# Autodesk Inventor assembly: Ensamblaje2
(part 2 of 3)
522. Tornillo Allen cabeza botón M4x10mm:7 — Insertar:733
523. Tornillo Allen cabeza botón M4x10mm:8 — Insertar:734
524. Tornillo Allen cabeza botón M4x20mm:43 — Insertar:747
525. Tornillo Allen cabeza botón M4x20mm:44 — Insertar:748
526. Tornillo Allen cabeza botón M4x20mm:45 — Insertar:750
527. Tornillo Allen cabeza botón M4x20mm:46 — Insertar:749
528. Tornillo Allen cabeza botón M4x20mm:47 — Insertar:739
529. Tornillo Allen cabeza botón M4x20mm:48 — Insertar:740
530. Tornillo Allen cabeza botón M4x20mm:49 — Insertar:741
531. Tornillo Allen cabeza botón M4x20mm:50 — Insertar:742
532. Arandela Plana Tipo A DIN 125 - M4:42 — Insertar:739, Insertar:743
533. Arandela Plana Tipo A DIN 125 - M4:43 — Insertar:740, Insertar:744
534. Arandela Plana Tipo A DIN 125 - M4:44 — Insertar:741, Insertar:745
535. Arandela Plana Tipo A DIN 125 - M4:45 — Insertar:742, Insertar:746
536. Puerta Frontal:1 — Coincidencia:409, Coincidencia:410, Insertar:826, Insertar:827, Insertar:842, Insertar:843, Insertar:844, Insertar:845, Ángulo:7
537. Puerta Lateral Derecha:1 — Insertar:755, Insertar:756, Insertar:806, Insertar:807, Insertar:808, Insertar:809, Insertar:810, Insertar:811, Ángulo:8
538. Puerta de Inspección:1 — Insertar:757, Coincidencia:407, Coincidencia:408, Insertar:800, Insertar:801, Insertar:802, Insertar:803, Insertar:804, Insertar:805, Ángulo:4
539. Tornillo Allen cabeza botón M4x10mm:15 — Insertar:764
540. Tornillo Allen cabeza botón M4x10mm:16 — Insertar:765
541. Tornillo Allen cabeza botón M4x10mm:17 — Insertar:766
542. Tornillo Allen cabeza botón M4x10mm:18 — Insertar:769
543. Tornillo Allen cabeza botón M4x10mm:19 — Insertar:768
544. Tornillo Allen cabeza botón M4x10mm:20 — Insertar:767
545. Tornillo Allen cabeza botón M4x10mm:23 — Insertar:772
546. Tornillo Allen cabeza botón M4x10mm:24 — Insertar:773
547. Tornillo Allen cabeza botón M4x10mm:25 — Insertar:775
548. Tornillo Allen cabeza botón M4x10mm:26 — Insertar:777
549. Tornillo Allen cabeza botón M4x10mm:27 — Insertar:776
550. Tornillo Allen cabeza botón M4x10mm:28 — Insertar:774
551. ISO 4032 M4:3 — Insertar:790
552. ISO 4032 M4:4 — Insertar:791
553. ISO 4032 M4:5 — Insertar:792
554. ISO 4032 M4:6 — Insertar:793
555. ISO 4032 M4:7 — Insertar:794
556. ISO 4032 M4:8 — Insertar:795
557. ISO 4032 M4:9 — Insertar:796
558. ISO 4032 M4:10 — Insertar:797
559. ISO 4032 M4:11 — Insertar:798
560. ISO 4032 M4:12 — Insertar:799
561. ISO 4032 M4:13 — Insertar:800
562. ISO 4032 M4:14 — Insertar:801
563. ISO 4032 M4:15 — Insertar:802
564. ISO 4032 M4:16 — Insertar:803
565. ISO 4032 M4:17 — Insertar:804
566. ISO 4032 M4:18 — Insertar:805
567. ISO 4032 M4:19 — Insertar:806
568. ISO 4032 M4:20 — Insertar:807
569. ISO 4032 M4:21 — Insertar:808
570. ISO 4032 M4:22 — Insertar:809
571. ISO 4032 M4:23 — Insertar:810
572. ISO 4032 M4:24 — Insertar:811
573. Arandela Plana Tipo A DIN 125 - M4:46 — Insertar:782, Insertar:797
574. Arandela Plana Tipo A DIN 125 - M4:47 — Insertar:781, Insertar:799
575. Arandela Plana Tipo A DIN 125 - M4:48 — Insertar:789, Insertar:795
576. Arandela Plana Tipo A DIN 125 - M4:49 — Insertar:780, Insertar:798
577. Arandela Plana Tipo A DIN 125 - M4:50 — Insertar:784, Insertar:790
578. Arandela Plana Tipo A DIN 125 - M4:51 — Insertar:785, Insertar:791
579. Arandela Plana Tipo A DIN 125 - M4:52 — Insertar:783, Insertar:796
580. Arandela Plana Tipo A DIN 125 - M4:53 — Insertar:786, Insertar:792
581. Arandela Plana Tipo A DIN 125 - M4:54 — Insertar:787, Insertar:793
582. Arandela Plana Tipo A DIN 125 - M4:55 — Insertar:788, Insertar:794
583. Tornillo allen cabeza boton M5x10mm:1 — Insertar:812
584. Tornillo allen cabeza boton M5x10mm:2 — Insertar:813
585. Tornillo allen cabeza boton M5x10mm:3 — Insertar:814
586. Tornillo allen cabeza boton M5x10mm:4 — Insertar:815
587. Soporte para culata carcasa:1 — Insertar:817, Insertar:818
588. Soporte para culata carcasa:2 — Insertar:816, Insertar:819
589. Tornillo Allen cabeza botón M4x10mm:55 — Insertar:829
590. Tornillo Allen cabeza botón M4x10mm:56 — Insertar:828
591. ISO 4032 M4:25 — Insertar:830
592. ISO 4032 M4:26 — Insertar:831
593. Tornillo Allen cabeza botón M4x16mm:1 — Insertar:840
594. Tornillo Allen cabeza botón M4x16mm:2 — Insertar:839
595. Tornillo Allen cabeza botón M4x16mm:3 — Insertar:838
596. Tornillo Allen cabeza botón M4x16mm:4 — Insertar:837
597. Tornillo Allen cabeza botón M4x16mm:5 — Insertar:836
598. Tornillo Allen cabeza botón M4x16mm:6 — Insertar:841
599. Tornillo Allen cabeza botón M4x16mm:7 — Insertar:832
600. Tornillo Allen cabeza botón M4x16mm:8 — Insertar:833
601. Tornillo Allen cabeza botón M4x16mm:9 — Insertar:834
602. Tornillo Allen cabeza botón M4x16mm:10 — Insertar:835
603. ISO 4032 M4:27 — Insertar:842
604. ISO 4032 M4:28 — Insertar:843
605. ISO 4032 M4:29 — Insertar:844
606. ISO 4032 M4:30 — Insertar:845
607. Tornillo Allen cabeeza botón M3x8mm:33 — Insertar:846, Coincidencia:415
608. Tornillo Allen cabeeza botón M3x8mm:34 — Insertar:847, Coincidencia:417
609. ISO 4032 M2:1 — Coincidencia:411, Coincidencia:412
610. ISO 4032 M2:2 — Coincidencia:413, Coincidencia:414
611. ISO 4032 M3:1 — Coincidencia:415, Coincidencia:416
612. ISO 4032 M3:2 — Coincidencia:417, Coincidencia:418
613. ISO 4032 M2:3 — Coincidencia:419, Coincidencia:420
614. ISO 4032 M2:4 — Coincidencia:421, Coincidencia:422
615. Kit de sujecion 2:2 — Insertar:854, Insertar:855, Insert:858, Insert:859
616. Kit sugecion 1:1 — Insertar:852, Insertar:853, Insert:856, Insert:857
617. Eslabon cadena portacable:1 — Coincidencia:423, Nivelación:60
618. Tornillo Allen cabeeza botón M3x8mm:35 — Insert:856
619. Tornillo Allen cabeeza botón M3x8mm:36 — Insert:857
620. Tornillo Allen cabeeza botón M3x16mm:1 — Insert:858
621. Tornillo Allen cabeeza botón M3x16mm:2 — Insert:859
622. ISO 4032 M3:3 — Insert:860
623. ISO 4032 M3:4 — Insert:861
## Relationships (824: Insert 566, Mate 220, Flush 35, Angle 3)
- Coincidencia:4 [Mate]: Culata:1 ↔ Lateral:1
- Insertar:1 (-20 mm): Soporte para Patas Regulables:4 ↔ Pata regulable M6:1
- Insertar:2 (-20 mm): Soporte para Patas Regulables:1 ↔ Pata regulable M6:2
- Insertar:3 (-20 mm): Soporte para Patas Regulables:2 ↔ Pata regulable M6:3
- Insertar:4 (-20 mm): Soporte para Patas Regulables:3 ↔ Pata regulable M6:4
- Coincidencia:21 [Mate]: Frente:1 ↔ Buje para Tornillo:1
- Coincidencia:22 [Mate]: Frente:1 ↔ Buje para Tornillo:1
- Coincidencia:37 [Mate]: Columna Izquierda:1 ↔ Travesaño Estructural:1
- Coincidencia:40 [Mate]: Columna Derecha:1 ↔ Travesaño Estructural:1
- Coincidencia:41 [Mate]: Columna Derecha:1 ↔ Travesaño Estructural:1
- Coincidencia:42 [Mate]: Columna Izquierda:1 ↔ Travesaño Estructural:1
- Coincidencia:43 [Mate]: Columna Izquierda:1 ↔ Travesaño Estructural:1
- Coincidencia:44 [Mate]: Columna Derecha:1 ↔ Travesaño Estructural:1
- Coincidencia:45 [Mate]: Columna Izquierda:1 ↔ Guías de Vínculo Cabezal:2
- Nivelación:7 [Flush]: Columna Derecha:1 ↔ Guías de Vínculo Cabezal:2
- Coincidencia:46 [Mate]: Columna Derecha:1 ↔ Guías de Vínculo Cabezal:1
- Nivelación:8 [Flush]: Columna Derecha:1 ↔ Guías de Vínculo Cabezal:1
- Coincidencia:47 [Mate]: Columna Izquierda:1 ↔ Buje para Tornillo:2
- Coincidencia:48 [Mate]: Columna Izquierda:1 ↔ Buje para Tornillo:2
- Insertar:17: Tornillo de Vínculo Cabezal:1 ↔ Buje para Tornillo:2
- Coincidencia:53 [Mate]: Vertical Vìnculo Cabezal:1 ↔ Piso, Vínculo Cabezal:1
- Coincidencia:54 [Mate]: Vertical Vìnculo Cabezal:1 ↔ Piso, Vínculo Cabezal:1
- Coincidencia:55 [Mate]: Vertical Vìnculo Cabezal:1 ↔ Techo, Vínculo Cabezal:1
- Coincidencia:56 [Mate]: Vertical Vìnculo Cabezal:1 ↔ Techo, Vínculo Cabezal:1
- Coincidencia:61 [Mate]: Guías de Vínculo Cabezal:2 ↔ Buje para Guía:8
- Coincidencia:62 [Mate]: Guías de Vínculo Cabezal:2 ↔ Buje para Guía:7
- Coincidencia:63 [Mate]: Guías de Vínculo Cabezal:2 ↔ Separador de Bujes:2
- Coincidencia:64 [Mate]: Guías de Vínculo Cabezal:1 ↔ Buje para Guía:5
- Coincidencia:65 [Mate]: Guías de Vínculo Cabezal:1 ↔ Separador de Bujes:1
- Coincidencia:66 [Mate]: Guías de Vínculo Cabezal:1 ↔ Buje para Guía:6
- Coincidencia:67 [Mate]: Buje para Guía:8 ↔ Separador de Bujes:2
- Coincidencia:68 [Mate]: Buje para Guía:7 ↔ Separador de Bujes:2
- Coincidencia:69 [Mate]: Buje para Guía:6 ↔ Separador de Bujes:1
- Coincidencia:70 [Mate]: Buje para Guía:5 ↔ Separador de Bujes:1
- Coincidencia:71 [Mate]: Guías de Vínculo Cabezal:2 ↔ Tapa para Buje:4
- Coincidencia:72 [Mate]: Guías de Vínculo Cabezal:2 ↔ Tapa para Buje:1
- Coincidencia:73 [Mate]: Guías de Vínculo Cabezal:1 ↔ Tapa para Buje:3
- Coincidencia:74 [Mate]: Guías de Vínculo Cabezal:1 ↔ Tapa para Buje:2
- Coincidencia:79 [Mate]: Piso, Vínculo Cabezal:1 ↔ Buje para Tornillo:3
- Coincidencia:80 [Mate]: Piso, Vínculo Cabezal:1 ↔ Buje para Tornillo:3
- Insertar:24: Buje para Tornillo:3 ↔ Tornillo de Soporte de Motor:1
- Insertar:35: Lateral:1 ↔ Tornillo allen cabeza cilindrica M6x20mm:16
- Insertar:36: Lateral:1 ↔ Tornillo allen cabeza cilindrica M6x20mm:17
- Insertar:37: Lateral:1 ↔ Tornillo allen cabeza cilindrica M6x20mm:15
- Insertar:38: Lateral:1 ↔ Tornillo allen cabeza cilindrica M6x20mm:10
- Insertar:71: Lateral:1 ↔ Soporte para Patas Regulables:4
- Insertar:72: Lateral:1 ↔ Soporte para Patas Regulables:1
- Coincidencia:89 [Mate]: Lateral:1 ↔ Soporte para Patas Regulables:4
- Coincidencia:90 [Mate]: Lateral:1 ↔ Soporte para Patas Regulables:1
- Insertar:73: Soporte para Patas Regulables:2 ↔ Tornillo Allen cabeza fresada M4x16mm:8
- Insertar:74: Soporte para Patas Regulables:2 ↔ Tornillo Allen cabeza fresada M4x16mm:4
- Insertar:75: Soporte para Patas Regulables:3 ↔ Tornillo Allen cabeza fresada M4x16mm:7
- Insertar:76: Soporte para Patas Regulables:3 ↔ Tornillo Allen cabeza fresada M4x16mm:6
- Insertar:77: Soporte para Patas Regulables:1 ↔ Tornillo Allen cabeza fresada M4x16mm:1
- Insertar:78: Soporte para Patas Regulables:1 ↔ Tornillo Allen cabeza fresada M4x16mm:2
- Insertar:79: Soporte para Patas Regulables:4 ↔ Tornillo Allen cabeza fresada M4x16mm:3
- Insertar:80: Soporte para Patas Regulables:4 ↔ Tornillo Allen cabeza fresada M4x16mm:5
- Insertar:82: Nema 17:1 ↔ Techo Espaciador Sub. Inferior:1
- Insertar:83: Tornillo Allen cabeza cilindrica M4x16mm:1 ↔ Techo Espaciador Sub. Inferior:1
- Insertar:84: Tornillo Allen cabeza cilindrica M4x16mm:3 ↔ Techo Espaciador Sub. Inferior:1
- Insertar:85: Tornillo Allen cabeza cilindrica M4x16mm:6 ↔ Techo Espaciador Sub. Inferior:1
- Insertar:86: Tornillo Allen cabeza cilindrica M4x16mm:2 ↔ Techo Espaciador Sub. Inferior:1
- Coincidencia:91 [Mate]: Culata:1 ↔ Espaciador Sub Inferior:2
- Coincidencia:92 [Mate]: Culata:1 ↔ Espaciador Sub Inferior:1
- Coincidencia:93 [Mate]: Culata:1 ↔ Espaciador Sub Inferior:1
- Coincidencia:94 [Mate]: Culata:1 ↔ Espaciador Sub Inferior:1
- Coincidencia:95 [Mate]: Culata:1 ↔ Espaciador Sub Inferior:2
- Coincidencia:96 [Mate]: Culata:1 ↔ Espaciador Sub Inferior:2
- Coincidencia:97 [Mate]: Espaciador Sub Inferior:1 ↔ Techo Espaciador Sub. Inferior:1
- Insertar:91: Espaciador Sub Inferior:1 ↔ Techo Espaciador Sub. Inferior:1
- Coincidencia:99 [Mate]: Tornillo Allen cabeza cilindrica M4x16mm:1 ↔ Nema 17:1
- Insertar:100: Arandela Grower m6:13 ↔ Tornillo Allen cabeza botón M6x20mm:3
- Insertar:103: Arandela Grower m6:9 ↔ Tornillo Allen cabeza botón M6x20mm:8
- Insertar:107: Arandela Grower m6:10 ↔ Tornillo Allen cabeza botón M6x20mm:4
- Insertar:109: Arandela Grower m6:7 ↔ Tornillo Allen cabeza botón M6x20mm:6
- Insertar:122: Arandela Grower m6:11 ↔ Tornillo Allen cabeza botón M6x20mm:11
- Insertar:123: Arandela Grower m6:14 ↔ Tornillo Allen cabeza botón M6x20mm:21
- Insertar:124: Arandela Grower m6:8 ↔ Tornillo Allen cabeza botón M6x20mm:12
- Insertar:125: Arandela Grower m6:12 ↔ Tornillo Allen cabeza botón M6x20mm:20
- Insertar:126: Columna Izquierda:1 ↔ Arandela Grower m6:14
- Insertar:127: Columna Izquierda:1 ↔ Arandela Grower m6:11
- Insertar:128: Columna Derecha:1 ↔ Arandela Grower m6:8
- Insertar:129: Columna Derecha:1 ↔ Arandela Grower m6:12
- Insertar:138: Vertical Vìnculo Cabezal:1 ↔ Tornillo Allen cabeza botón M6x20mm:18
- Insertar:139: Vertical Vìnculo Cabezal:1 ↔ Tornillo Allen cabeza botón M6x20mm:25
- Insertar:140: Vertical Vìnculo Cabezal:1 ↔ Tornillo Allen cabeza botón M6x20mm:24
- Insertar:141: Vertical Vìnculo Cabezal:1 ↔ Tornillo Allen cabeza botón M6x20mm:28
- Insertar:142: Vertical Vìnculo Cabezal:1 ↔ Tornillo Allen cabeza botón M6x20mm:27
- Insertar:143: Vertical Vìnculo Cabezal:1 ↔ Tornillo Allen cabeza botón M6x20mm:23
- Insertar:144: Vertical Vìnculo Cabezal:1 ↔ Tornillo Allen cabeza botón M6x20mm:22
- Insertar:145: Vertical Vìnculo Cabezal:1 ↔ Tornillo Allen cabeza botón M6x20mm:26
- Insertar:148: Tapa para Buje:1 ↔ Tornillo Allen cabeeza botón M3x8mm:7
- Insertar:149: Tapa para Buje:1 ↔ Tornillo Allen cabeeza botón M3x8mm:8
- Insertar:150: Tapa para Buje:3 ↔ Tornillo Allen cabeeza botón M3x8mm:2
- Insertar:151: Tapa para Buje:3 ↔ Tornillo Allen cabeeza botón M3x8mm:6
- Insertar:152: Tapa para Buje:4 ↔ Tornillo Allen cabeeza botón M3x8mm:3
- Insertar:153: Tapa para Buje:4 ↔ Tornillo Allen cabeeza botón M3x8mm:1
- Insertar:154: Tapa para Buje:2 ↔ Tornillo Allen cabeeza botón M3x8mm:4
- Insertar:155: Tapa para Buje:2 ↔ Tornillo Allen cabeeza botón M3x8mm:5
- Coincidencia:105 [Mate]: Techo, Vínculo Cabezal:1 ↔ Espaciador Izquierdo:1
- Coincidencia:106 [Mate]: Techo, Vínculo Cabezal:1 ↔ Espaciador Izquierdo:1
- Coincidencia:107 [Mate]: Techo, Vínculo Cabezal:1 ↔ Espaciador Izquierdo:1
- Coincidencia:108 [Mate]: Techo, Vínculo Cabezal:1 ↔ Espaciador Derecho:1
- Coincidencia:109 [Mate]: Techo, Vínculo Cabezal:1 ↔ Espaciador Derecho:1
- Coincidencia:110 [Mate]: Techo, Vínculo Cabezal:1 ↔ Espaciador Derecho:1
- Coincidencia:111 [Mate]: Espaciador Izquierdo:1 ↔ Techo Espaciador:1
- Coincidencia:112 [Mate]: Espaciador Derecho:1 ↔ Techo Espaciador:1
- Coincidencia:113 [Mate]: Espaciador Derecho:1 ↔ Techo Espaciador:1
- Coincidencia:114 [Mate]: Espaciador Izquierdo:1 ↔ Techo Espaciador:1
- Coincidencia:115 [Mate]: Nema 17:3 ↔ Acople de Motor PAP:3
- Insertar:165: Techo Espaciador:1 ↔ Tornillo Allen cabeza cilindrica M4x20mm:3
- Insertar:166: Techo Espaciador:1 ↔ Tornillo Allen cabeza cilindrica M4x20mm:2
- Insertar:167: Techo Espaciador:1 ↔ Tornillo Allen cabeza cilindrica M4x20mm:1
- Insertar:168: Techo Espaciador:1 ↔ Tornillo Allen cabeza cilindrica M4x20mm:4
- Insertar:169: Nema 17:3 ↔ Techo Espaciador:1
- Insertar:170: Columna Derecha:1 ↔ Tornillo Allen cabeza botón M4x20mm:5
- Insertar:172: Columna Derecha:1 ↔ Tornillo Allen cabeza botón M4x20mm:4
- Insertar:173: Columna Derecha:1 ↔ Tornillo Allen cabeza botón M4x20mm:3
- Coincidencia:116 [Mate]: Columna Derecha:1 ↔ Nema 17:2
- Insertar:174: Columna Derecha:1 ↔ Nema 17:2
- Insertar:175: Columna Derecha:1 ↔ Nema 17:2
- Coincidencia:117 [Mate]: Tornillo de Vínculo Cabezal:1 ↔ Nema 17:2
- Insertar:176: Tornillo de Vínculo Cabezal:1 ↔ Acople de Motor PAP:2
- Coincidencia:118 [Mate]: Vertical Vìnculo Cabezal:1 ↔ Bloque - Vinculo Cabezal:1
- Coincidencia:119 [Mate]: Bloque - Vinculo Cabezal:1 ↔ Techo, Vínculo Cabezal:1
- Coincidencia:120 [Mate]: Vertical Vìnculo Cabezal:1 ↔ Bloque - Vinculo Cabezal:1
- Insertar:177: Bloque - Vinculo Cabezal:1 ↔ Buje para Guía:7
- Insertar:178: Bloque - Vinculo Cabezal:1 ↔ Buje para Guía:5
- Insertar:179: Bloque - Vinculo Cabezal:1 ↔ Tapa para Buje:4
- Insertar:180: Bloque - Vinculo Cabezal:1 ↔ Tapa para Buje:2
- Insertar:181: Bloque - Vinculo Cabezal:1 ↔ Tapa para Buje:1
- Insertar:182: Bloque - Vinculo Cabezal:1 ↔ Tapa para Buje:3
- Insertar:185: Techo Espaciador:1 ↔ Tornillo Allen cabeza cilindrica M4x45mm:3
- Insertar:186: Techo Espaciador:1 ↔ Tornillo Allen cabeza cilindrica M4x45mm:1
- Insertar:187: Techo Espaciador:1 ↔ Tornillo Allen cabeza cilindrica M4x45mm:4
- Coincidencia:125 [Mate]: Bloque - Vinculo Cabezal:1 ↔ Acople de Motor PAP:2
- Coincidencia:126 [Mate]: Columna Izquierda:1 ↔ Soporte de Final de Carrera - Eje X:1
- Coincidencia:127 [Mate]: Columna Izquierda:1 ↔ Soporte de Final de Carrera - Eje X:1
- Coincidencia:128 [Mate]: Columna Izquierda:1 ↔ Soporte de Final de Carrera - Eje X:1
- Coincidencia:129 [Mate]: Final de Carrera:2 ↔ Soporte de Final de Carrera - Eje X:1
- Coincidencia:130 [Mate]: Final de Carrera:2 ↔ Soporte de Final de Carrera - Eje X:1
- Coincidencia:131 [Mate]: Final de Carrera:2 ↔ Soporte de Final de Carrera - Eje X:1
- Coincidencia:139 [Mate]: Bloque - Vinculo Cabezal:1 ↔ Final de Carrera:2
- Insertar:201: Columna Izquierda:1 ↔ Arandela Grower m6:21
- Insertar:202: Columna Izquierda:1 ↔ Arandela Grower m6:20
- Insertar:203: Columna Izquierda:1 ↔ Arandela Grower m6:19
- Insertar:204: Columna Izquierda:1 ↔ Arandela Grower m6:24
- Insertar:205: Columna Derecha:1 ↔ Arandela Grower m6:23
- Insertar:206: Columna Derecha:1 ↔ Arandela Grower m6:17
- Insertar:207: Columna Derecha:1 ↔ Arandela Grower m6:22
- Insertar:208: Columna Derecha:1 ↔ Arandela Grower m6:18
- Insertar:213: Soporte de Final de Carrera - Eje X:1 ↔ Tornillo Allen cabeeza botón M3x8mm:10
- Insertar:214: Soporte de Final de Carrera - Eje X:1 ↔ Tornillo Allen cabeeza botón M3x8mm:9
- Insertar:217: Techo Espaciador:1 ↔ Tornillo Allen cabeza cilindrica M4x45mm:4
- Insertar:218: Techo Espaciador:1 ↔ Tornillo Allen cabeza cilindrica M4x45mm:1
- Insertar:219: Techo Espaciador:1 ↔ Tornillo Allen cabeza cilindrica M4x45mm:2
- Insertar:220: Techo Espaciador:1 ↔ Tornillo Allen cabeza cilindrica M4x45mm:3
- Coincidencia:148 [Mate]: Culata:1 ↔ Tornillo allen cabeza cilindrica M6x20mm:15
- Nivelación:12 [Flush]: Frente:1 ↔ Lateral:1
- Nivelación:16 [Flush]: Frente:1 ↔ Lateral:2
- Nivelación:17 [Flush]: Frente:1 ↔ Lateral:2
- Coincidencia:154 [Mate]: Frente:1 ↔ Lateral:2
- Insertar:234: Lateral:2 ↔ Tornillo allen cabeza cilindrica M6x20mm:20
- Insertar:235: Lateral:2 ↔ Tornillo allen cabeza cilindrica M6x20mm:5
- Insertar:236: Frente:1 ↔ Lateral:1
- Insertar:237: Lateral:2 ↔ Columna Derecha:1
- Insertar:238: Lateral:2 ↔ Columna Derecha:1
- Insertar:239: Lateral:2 ↔ Soporte para Patas Regulables:2
- Coincidencia:155 [Mate]: Lateral:2 ↔ Tornillo Allen cabeza fresada M4x16mm:4
- Insertar:254: Lateral:2 ↔ Soporte para Patas Regulables:3
- Coincidencia:170 [Mate]: Lateral:2 ↔ Soporte para Patas Regulables:3
- Coincidencia:171 [Mate]: Bloque - Vinculo Cabezal:1 ↔ Tornillo Gusano Allen M3x16mm:1
- Coincidencia:172 [Mate]: Bloque - Vinculo Cabezal:1 ↔ Tornillo Gusano Allen M3x16mm:2
- Coincidencia:173 [Mate]: Tornillo de Vínculo Cabezal:1 ↔ Tuerca de mesa:3
- Insertar:255 (10 mm): Bloque - Vinculo Cabezal:1 ↔ Tuerca de mesa:3
- Coincidencia:174 [Mate]: Bloque - Vinculo Cabezal:1 ↔ Tuerca de mesa:3
- Nivelación:18 [Flush]: Tornillo Gusano Allen M3x16mm:1 ↔ Tuerca de mesa:3
- Nivelación:19 [Flush]: Tornillo Gusano Allen M3x16mm:2 ↔ Tuerca de mesa:3
- Insertar:257: Tornillo Gusano Allen M3x16mm:4 ↔ Tuerca de mesa:2
- Coincidencia:180 [Mate]: Guías de Soporte de Motor:1 ↔ Buje de Soporte de Motor:2
- Insertar:266: Buje de Soporte de Motor:1 ↔ Tornillo Allen cabeeza botón M3x8mm:11
- Coincidencia:182 [Mate]: Guías de Soporte de Motor:2 ↔ Buje de Soporte de Motor:5
- Insertar:268: Buje de Soporte de Motor:2 ↔ Tornillo Allen cabeeza botón M3x8mm:13
- Insertar:270: Tornillo Allen cabeeza botón M3x8mm:12 ↔ Buje de Soporte de Motor:6
- Insertar:271: Buje de Soporte de Motor:5 ↔ Tornillo Allen cabeeza botón M3x8mm:16
- Nivelación:20 [Flush]: Culata:1 ↔ Acople de Motor PAP:1
- Coincidencia:186 [Mate]: Culata:1 ↔ Acople de Motor PAP:1
- Insertar:278: Tornillo de mesa:1 ↔ Buje para Tornillo:1
- Insertar:279: Techo, Vínculo Cabezal:1 ↔ Guías de Soporte de Motor:2
- Insertar:280: Techo, Vínculo Cabezal:1 ↔ Guías de Soporte de Motor:1
- Insertar:285: Frente:1 ↔ Guias de mesa:1
- Coincidencia:190 [Mate]: Guias de mesa:1 ↔ Buje para Guía:2
- Coincidencia:193 [Mate]: Frente:1 ↔ Guias de mesa:2
- Insertar:286: Frente:1 ↔ Guias de mesa:2
- Coincidencia:194 [Mate]: Guias de mesa:2 ↔ Buje para Guía:4
- Coincidencia:197 [Mate]: Mesa:1 ↔ Soporte de Buje:4
- Coincidencia:198 [Mate]: Mesa:1 ↔ Soporte de Buje:3
- Coincidencia:200 [Mate]: Mesa:1 ↔ Soporte de Buje:4
- Coincidencia:203 [Mate]: Mesa:1 ↔ Soporte de Buje:3
- Coincidencia:205 [Mate]: Mesa:1 ↔ Soporte de Buje:4
- Coincidencia:206 [Mate]: Mesa:1 ↔ Soporte de Buje:3
- Coincidencia:208 [Mate]: Mesa:1 ↔ Soporte de tuerca de mesa:1
- Coincidencia:209 [Mate]: Mesa:1 ↔ Soporte de tuerca de mesa:1
- Coincidencia:210 [Mate]: Mesa:1 ↔ Soporte de tuerca de mesa:1
- Coincidencia:211 [Mate]: Soporte de Buje:1 ↔ Buje para Guía:2
- Coincidencia:212 [Mate]: Guias de mesa:1 ↔ Buje para Guía:1
- Coincidencia:213 [Mate]: Soporte de Buje:2 ↔ Buje para Guía:1
- Nivelación:21 [Flush]: Soporte de Buje:2 ↔ Buje para Guía:1
- Nivelación:22 [Flush]: Soporte de Buje:1 ↔ Buje para Guía:2
- Coincidencia:214 [Mate]: Soporte de Buje:4 ↔ Buje para Guía:4
- Nivelación:23 [Flush]: Soporte de Buje:4 ↔ Buje para Guía:4
- Coincidencia:215 [Mate]: Soporte de Buje:3 ↔ Buje para Guía:3
- Nivelación:24 [Flush]: Soporte de Buje:3 ↔ Buje para Guía:3
- Coincidencia:216 [Mate]: Tornillo de mesa:1 ↔ Soporte de tuerca de mesa:1
- Coincidencia:217 [Mate]: Mesa:1 ↔ Soporte de Buje:2
- Coincidencia:218 [Mate]: Mesa:1 ↔ Soporte de Buje:1
- Insertar:287: Soporte de Buje:3 ↔ Tornillo Allen cabeza cilindrica M4x30mm:6
- Insertar:288: Soporte de Buje:3 ↔ Tornillo Allen cabeza cilindrica M4x30mm:9
- Insertar:289: Soporte de Buje:3 ↔ Tornillo Allen cabeza cilindrica M4x30mm:18
- Insertar:290: Soporte de Buje:3 ↔ Tornillo Allen cabeza cilindrica M4x30mm:1
- Insertar:291: Soporte de Buje:2 ↔ Tornillo Allen cabeza cilindrica M4x30mm:2
- Insertar:292: Soporte de Buje:2 ↔ Tornillo Allen cabeza cilindrica M4x30mm:16
- Insertar:293: Soporte de Buje:2 ↔ Tornillo Allen cabeza cilindrica M4x30mm:15
- Insertar:294: Soporte de Buje:2 ↔ Tornillo Allen cabeza cilindrica M4x30mm:7
- Insertar:295: Soporte de Buje:4 ↔ Tornillo Allen cabeza cilindrica M4x30mm:20
- Insertar:296: Soporte de Buje:4 ↔ Tornillo Allen cabeza cilindrica M4x30mm:17
- Insertar:297: Soporte de Buje:4 ↔ Tornillo Allen cabeza cilindrica M4x30mm:19
- Insertar:298: Soporte de Buje:4 ↔ Tornillo Allen cabeza cilindrica M4x30mm:5
- Insertar:299: Soporte de Buje:1 ↔ Tornillo Allen cabeza cilindrica M4x30mm:3
- Insertar:300: Soporte de Buje:1 ↔ Tornillo Allen cabeza cilindrica M4x30mm:10
- Insertar:301: Soporte de Buje:1 ↔ Tornillo Allen cabeza cilindrica M4x30mm:4
- Insertar:302: Soporte de Buje:1 ↔ Tornillo Allen cabeza cilindrica M4x30mm:8
- Insertar:303: Soporte de tuerca de mesa:1 ↔ Tornillo Allen cabeza cilindrica M4x16mm:5
- Insertar:304: Soporte de tuerca de mesa:1 ↔ Tornillo Allen cabeza cilindrica M4x16mm:8
- Insertar:305: Soporte de tuerca de mesa:1 ↔ Tornillo Allen cabeza cilindrica M4x16mm:7
- Insertar:306: Soporte de tuerca de mesa:1 ↔ Tornillo Allen cabeza cilindrica M4x16mm:4
- Insertar:307 (10 mm): Soporte de tuerca de mesa:1 ↔ Tuerca de mesa:2
- Coincidencia:219 [Mate]: Soporte de tuerca de mesa:1 ↔ Tornillo Gusano Allen M3x16mm:4
- Insertar:308: Lateral:2 ↔ Tornillo allen cabeza cilindrica M6x20mm:7
- Coincidencia:220 [Mate]: Culata:1 ↔ Tornillo allen cabeza cilindrica M6x20mm:7
- Insertar:320: Arandela Grower m6:1 ↔ Arandela plana tipo A DIN 125 M6:8
- Insertar:322: Arandela Grower m6:2 ↔ Arandela plana tipo A DIN 125 M6:7
- Insertar:323: Guias de mesa:2 ↔ Arandela plana tipo A DIN 125 M6:7
- Insertar:324: Guias de mesa:1 ↔ Arandela plana tipo A DIN 125 M6:8
- Insertar:326: Arandela Grower m6:3 ↔ Arandela plana tipo A DIN 125 M6:3
- Insertar:328: Arandela Grower m6:4 ↔ Arandela plana tipo A DIN 125 M6:2
- Insertar:329: Guias de mesa:2 ↔ Arandela plana tipo A DIN 125 M6:2
- Insertar:330: Guias de mesa:1 ↔ Arandela plana tipo A DIN 125 M6:3
- Insertar:331: Arandela Grower m6:7 ↔ Arandela plana tipo A DIN 125 M6:1
- Insertar:332: Guías de Vínculo Cabezal:2 ↔ Arandela plana tipo A DIN 125 M6:1
- Insertar:333: Arandela Grower m6:10 ↔ Arandela plana tipo A DIN 125 M6:4
- Insertar:334: Guías de Vínculo Cabezal:1 ↔ Arandela plana tipo A DIN 125 M6:4
- Insertar:335: Arandela Grower m6:13 ↔ Arandela plana tipo A DIN 125 M6:5
- Insertar:336: Guías de Vínculo Cabezal:2 ↔ Arandela plana tipo A DIN 125 M6:5
- Insertar:337: Arandela Grower m6:9 ↔ Arandela plana tipo A DIN 125 M6:6
- Insertar:338: Guías de Vínculo Cabezal:1 ↔ Arandela plana tipo A DIN 125 M6:6
- Insertar:340: Buje para Guía:4 ↔ Tapa para Buje:7
- Insertar:341: Buje para Guía:1 ↔ Tapa para Buje:9
- Insertar:342: Buje para Guía:3 ↔ Tapa para Buje:6
- Insertar:343: Buje para Guía:3 ↔ Tapa para Buje:8
- Insertar:344: Buje para Guía:1 ↔ Tapa para Buje:10
- Insertar:345: Buje para Guía:4 ↔ Tapa para Buje:12
- Insertar:346: Buje para Guía:2 ↔ Tapa para Buje:11
- Coincidencia:250 [Mate]: Soporte de Buje:4 ↔ Tapa para Buje:7
- Insertar:347: Tapa para Buje:7 ↔ Tornillo Allen cabeeza botón M3x8mm:17
- Insertar:348: Tapa para Buje:7 ↔ Tornillo Allen cabeeza botón M3x8mm:25
- Insertar:349: Buje para Guía:2 ↔ Tapa para Buje:5
- Coincidencia:251 [Mate]: Soporte de Buje:1 ↔ Tapa para Buje:5
- Coincidencia:252 [Mate]: Soporte de Buje:2 ↔ Tapa para Buje:9
- Coincidencia:253 [Mate]: Soporte de Buje:3 ↔ Tapa para Buje:6
- Coincidencia:254 [Mate]: Soporte de Buje:2 ↔ Tapa para Buje:10
- Coincidencia:255 [Mate]: Soporte de Buje:3 ↔ Tapa para Buje:8
- Coincidencia:256 [Mate]: Soporte de Buje:1 ↔ Tapa para Buje:11
- Coincidencia:257 [Mate]: Soporte de Buje:4 ↔ Tapa para Buje:12
- Insertar:350: Tapa para Buje:5 ↔ Tornillo Allen cabeeza botón M3x8mm:32
- Insertar:351: Tapa para Buje:5 ↔ Tornillo Allen cabeeza botón M3x8mm:31
- Insertar:352: Tapa para Buje:9 ↔ Tornillo Allen cabeeza botón M3x8mm:30
- Insertar:353: Tapa para Buje:6 ↔ Tornillo Allen cabeeza botón M3x8mm:29
- Insertar:354: Tapa para Buje:9 ↔ Tornillo Allen cabeeza botón M3x8mm:22
- Insertar:355: Tapa para Buje:6 ↔ Tornillo Allen cabeeza botón M3x8mm:21
- Insertar:356: Tapa para Buje:10 ↔ Tornillo Allen cabeeza botón M3x8mm:20
- Insertar:357: Tapa para Buje:10 ↔ Tornillo Allen cabeeza botón M3x8mm:28
- Insertar:358: Tapa para Buje:8 ↔ Tornillo Allen cabeeza botón M3x8mm:27
- Insertar:359: Tapa para Buje:8 ↔ Tornillo Allen cabeeza botón M3x8mm:26
- Insertar:360: Tapa para Buje:11 ↔ Tornillo Allen cabeeza botón M3x8mm:24
- Insertar:361: Tapa para Buje:12 ↔ Tornillo Allen cabeeza botón M3x8mm:23
- Insertar:362: Tapa para Buje:12 ↔ Tornillo Allen cabeeza botón M3x8mm:19
- Insertar:363: Tapa para Buje:11 ↔ Tornillo Allen cabeeza botón M3x8mm:18
- Insertar:364: Techo, Vínculo Cabezal:1 ↔ Tornillo Allen cabeza botón M6x16mm:4
- Insertar:365: Techo, Vínculo Cabezal:1 ↔ Tornillo Allen cabeza botón M6x16mm:3
- Insertar:366: Techo, Vínculo Cabezal:1 ↔ Tornillo Allen cabeza botón M6x16mm:2
- Insertar:367: Techo, Vínculo Cabezal:1 ↔ Tornillo Allen cabeza botón M6x16mm:1
- Insertar:368: Piso, Vínculo Cabezal:1 ↔ Tornillo Allen cabeza botón M6x16mm:8
- Insertar:369: Piso, Vínculo Cabezal:1 ↔ Tornillo Allen cabeza botón M6x16mm:7
- Insertar:370: Piso, Vínculo Cabezal:1 ↔ Tornillo Allen cabeza botón M6x16mm:6
- Insertar:371: Piso, Vínculo Cabezal:1 ↔ Tornillo Allen cabeza botón M6x16mm:5
- Insertar:372: Arandela Grower m6:5 ↔ Tornillo Allen cabeza botón M6x20mm:7
- Insertar:373: Arandela Grower m6:5 ↔ Arandela plana tipo A DIN 125 M6:10
- Insertar:374: Arandela Grower m6:6 ↔ Tornillo Allen cabeza botón M6x20mm:5
- Insertar:375: Arandela Grower m6:6 ↔ Arandela plana tipo A DIN 125 M6:9
- Insertar:376: Arandela Grower m6:16 ↔ Tornillo Allen cabeza botón M6x20mm:9
- Insertar:377: Arandela Grower m6:16 ↔ Arandela plana tipo A DIN 125 M6:11
- Insertar:378: Arandela Grower m6:15 ↔ Tornillo Allen cabeza botón M6x20mm:10
- Insertar:379: Arandela Grower m6:15 ↔ Arandela plana tipo A DIN 125 M6:12
- Insertar:380: Guías de Soporte de Motor:2 ↔ Arandela plana tipo A DIN 125 M6:9
- Insertar:381: Guías de Soporte de Motor:1 ↔ Arandela plana tipo A DIN 125 M6:10
- Insertar:382: Guías de Soporte de Motor:2 ↔ Arandela plana tipo A DIN 125 M6:11
- Insertar:383: Guías de Soporte de Motor:1 ↔ Arandela plana tipo A DIN 125 M6:12
- Coincidencia:258 [Mate]: Guías de Soporte de Motor:2 ↔ Buje de Soporte de Motor:1
- Coincidencia:259 [Mate]: Guías de Soporte de Motor:1 ↔ Buje de Soporte de Motor:6
- Insertar:385: Tornillo allen cabeza boton M8x16mm:4 ↔ Arandela Grower M8:4
- Insertar:386: Tornillo allen cabeza boton M8x16mm:3 ↔ Arandela Grower M8:1
- Insertar:387: Tornillo allen cabeza boton M8x16mm:2 ↔ Arandela Grower M8:2
- Insertar:388: Tornillo allen cabeza boton M8x16mm:1 ↔ Arandela Grower M8:3
- Coincidencia:263 [Mate]: Acople de soporte de motor:1 ↔ Guías de Soporte de Motor:1
- Coincidencia:264 [Mate]: Acople de soporte de motor:1 ↔ Guías de Soporte de Motor:2
- Insertar:389: Acople de soporte de motor:1 ↔ Buje de Soporte de Motor:5
- Coincidencia:265 [Mate]: Acople de soporte de motor:1 ↔ Tornillo Allen cabeeza botón M3x8mm:16
- Insertar:390: Acople de soporte de motor:1 ↔ Buje de Soporte de Motor:2
- Coincidencia:266 [Mate]: Acople de soporte de motor:1 ↔ Tornillo Allen cabeeza botón M3x8mm:13
- Insertar:391: Acople de soporte de motor:1 ↔ Buje de Soporte de Motor:1
- Coincidencia:267 [Mate]: Acople de soporte de motor:1 ↔ Tornillo Allen cabeeza botón M3x8mm:11
- Insertar:392: Acople de soporte de motor:1 ↔ Buje de Soporte de Motor:6
- Coincidencia:268 [Mate]: Acople de soporte de motor:1 ↔ Tornillo Allen cabeeza botón M3x8mm:12
- Insertar:393: Acople de soporte de motor:1 ↔ Arandela Grower M8:1
- Insertar:394: Acople de soporte de motor:1 ↔ Arandela Grower M8:2
- Insertar:395: Acople de soporte de motor:1 ↔ Arandela Grower M8:3
- Insertar:396: Acople de soporte de motor:1 ↔ Arandela Grower M8:4
- Insertar:397: Acople de soporte de motor:1 ↔ Soporte de Motor:1
- Coincidencia:269 [Mate]: Soporte de Motor:1 ↔ Tornillo allen cabeza boton M8x16mm:2
- Coincidencia:270 [Mate]: motor DC:1 ↔ Soporte de Motor:1
- Nivelación:31 [Flush] (-3 mm): motor DC:1 ↔ Soporte de Motor:1
- Coincidencia:271 [Mate] (5 mm): Techo, Vínculo Cabezal:1 ↔ Buje de Soporte de Motor:5
- Coincidencia:272 [Mate]: Piso, Vínculo Cabezal:1 ↔ Buje de Soporte de Motor:1
- Coincidencia:273 [Mate]: motor DC:1 ↔ Herramienta Punta de Lanza:1
- Nivelación:32 [Flush] (-12 mm): motor DC:1 ↔ Herramienta Punta de Lanza:1
- Coincidencia:274 [Mate]: Frente:1 ↔ Mesa:1
- Mate:275: Culata:1 ↔ Mesa:1
- Insertar:398: Final de Carrera:1 ↔ Soporte de Final de Carrera - Eje Y:1
- Coincidencia:277 [Mate]: Final de Carrera:1 ↔ Soporte de Final de Carrera - Eje Y:1
- Coincidencia:279 [Mate]: Placa de Mecanizado:1 ↔ placa pcb 100x150mm:1
- Nivelación:34 [Flush]: Placa de Mecanizado:1 ↔ placa pcb 100x150mm:1
- Nivelación:35 [Flush]: Placa de Mecanizado:1 ↔ placa pcb 100x150mm:1
- Nivelación:36 [Flush] (50 mm): Mesa:1 ↔ Placa de Mecanizado:1
- Coincidencia:280 [Mate]: Mesa:1 ↔ Placa de Mecanizado:1
- Nivelación:37 [Flush] (30 mm): Mesa:1 ↔ Placa de Mecanizado:1
- Coincidencia:290 [Mate]: Tornillo de Soporte de Motor:1 ↔ Nema 17:3
- Insertar:410 (-12 mm): Tornillo de Soporte de Motor:1 ↔ Acople de Motor PAP:3
- Insertar:411: Techo, Vínculo Cabezal:1 ↔ Final de Carrera:3
- Coincidencia:291 [Mate]: Techo, Vínculo Cabezal:1 ↔ Final de Carrera:3
- Nivelación:38 [Flush]: Culata:1 ↔ Soporte de Final de Carrera - Eje Y:1
- Coincidencia:292 [Mate]: Culata:1 ↔ Soporte de Final de Carrera - Eje Y:1
- Nivelación:39 [Flush] (100 mm): Lateral:1 ↔ Soporte de Final de Carrera - Eje Y:1
- Insert:412: Techo Espaciador Sub. Inferior:1 ↔ Tornillo Allen cabeza cilindrica M4x35mm:1
- Insert:413: Techo Espaciador Sub. Inferior:1 ↔ Tornillo Allen cabeza cilindrica M4x35mm:4
- Insert:414: Techo Espaciador Sub. Inferior:1 ↔ Tornillo Allen cabeza cilindrica M4x35mm:3
- Insert:415: Techo Espaciador Sub. Inferior:1 ↔ Tornillo Allen cabeza cilindrica M4x35mm:2
- Mate:293: Espaciador Sub Inferior:2 ↔ Tornillo Allen cabeza cilindrica M4x35mm:2
- Insert:416: Final de Carrera:3 ↔ Tornillo Allen cabeza cilindrica M2x16mm:2
- Insert:417: Final de Carrera:3 ↔ Tornillo Allen cabeza cilindrica M2x16mm:1
- Insert:418: Final de Carrera:2 ↔ Tornillo Allen cabeza cilindrica M2x16mm:3
- Insert:419: Final de Carrera:2 ↔ Tornillo Allen cabeza cilindrica M2x16mm:4
- Insert:420: Final de Carrera:1 ↔ Tornillo Allen cabeza cilindrica M2x16mm:6
- Insert:421: Final de Carrera:1 ↔ Tornillo Allen cabeza cilindrica M2x16mm:7
- Mate:294 (-9 mm): motor DC:1 ↔ Tapa de Mandril:1
- Mate:295: motor DC:1 ↔ Tapa de Mandril:1
- Insert:422: Arandela Grower m6:21 ↔ Tornillo Allen cabeza botón M6x20mm:37
- Insert:423: Arandela Grower m6:24 ↔ Tornillo Allen cabeza botón M6x20mm:38
- Insert:424: Arandela Grower m6:19 ↔ Tornillo Allen cabeza botón M6x20mm:39
- Insert:425: Arandela Grower m6:20 ↔ Tornillo Allen cabeza botón M6x20mm:40
- Insert:426: Arandela Grower m6:4 ↔ Tornillo Allen cabeza botón M6x20mm:30
- Insert:427: Arandela Grower m6:3 ↔ Tornillo Allen cabeza botón M6x20mm:29
- Insert:428: Arandela Grower m6:2 ↔ Tornillo Allen cabeza botón M6x20mm:32
- Insert:429: Arandela Grower m6:1 ↔ Tornillo Allen cabeza botón M6x20mm:31
- Insert:430: Arandela Grower m6:22 ↔ Tornillo Allen cabeza botón M6x20mm:33
- Insert:431: Arandela Grower m6:23 ↔ Tornillo Allen cabeza botón M6x20mm:34
- Insert:432: Arandela Grower m6:17 ↔ Tornillo Allen cabeza botón M6x20mm:36
- Insert:433: Arandela Grower m6:18 ↔ Tornillo Allen cabeza botón M6x20mm:35
- Insert:442: Columna Derecha:1 ↔ Tornillo Allen cabeza botón M4x20mm:6
- Flush:40: Soporte de Motor:1 ↔ Tornillo Allen gusano M6 para Motor:1
- Mate:296: Soporte de Motor:1 ↔ Tornillo Allen gusano M6 para Motor:1
- Mate:301: Lateral:1 ↔ Guía de Bandeja Izq.:1
- Mate:302: Lateral:1 ↔ Guía de Bandeja Izq.:1
- Mate:303: Lateral:1 ↔ Guía de Bandeja Izq.:1
- Mate:304: Lateral:2 ↔ Guía de Bandeja Der.:1
- Mate:305: Lateral:2 ↔ Guía de Bandeja Der.:1
- Mate:306: Lateral:2 ↔ Guía de Bandeja Der.:1
- Insert:443: Guía de Bandeja Izq.:1 ↔ Tornillo Allen cabeza botón M4x10mm:4
- Insert:444: Guía de Bandeja Izq.:1 ↔ Tornillo Allen cabeza botón M4x10mm:6
- Insert:445: Guía de Bandeja Izq.:1 ↔ Tornillo Allen cabeza botón M4x10mm:5
- Insert:446: Guía de Bandeja Der.:1 ↔ Tornillo Allen cabeza botón M4x10mm:3
- Insert:447: Guía de Bandeja Der.:1 ↔ Tornillo Allen cabeza botón M4x10mm:2
- Insert:448: Guía de Bandeja Der.:1 ↔ Tornillo Allen cabeza botón M4x10mm:1
- Mate:307: Esquina de bandeja:1 ↔ Bandeja:1
- Mate:308: Esquina de bandeja:1 ↔ Bandeja:1
- Mate:309 (0.5 mm): Esquina de bandeja:1 ↔ Bandeja:1
- Mate:311: Esquina de bandeja:1 ↔ Bandeja:1
- Mate:312 (0.5 mm): Bandeja:1 ↔ Esquina de bandeja:2
- Mate:319: Bandeja:1 ↔ Esquina de bandeja:2
- Mate:320: Bandeja:1 ↔ Esquina de bandeja:2
- Mate:321: Bandeja:1 ↔ Esquina de bandeja:2
- Insert:449: Remache POP Abierto con Rotura de Vástago D4:8 ↔ Bandeja:1
- Insert:451: Remache POP Abierto con Rotura de Vástago D4:6 ↔ Bandeja:1
- Mate:331: Bandeja:1 ↔ Esquina de bandeja:3
- Mate:333: Bandeja:1 ↔ Esquina de bandeja:4
- Insert:454: Bandeja:1 ↔ Remache POP Abierto con Rotura de Vástago D4:10
- Insert:455: Bandeja:1 ↔ Remache POP Abierto con Rotura de Vástago D4:12
- Mate:337: Bandeja:1 ↔ Esquina de bandeja:2
- Mate:338: Bandeja:1 ↔ Esquina de bandeja:3
- Mate:339: Bandeja:1 ↔ Esquina de bandeja:4
- Mate:340: Esquina de bandeja:1 ↔ Bandeja:1
- Insert:456: Remache POP Abierto con Rotura de Vástago D4:7 ↔ Bandeja:1
- Insert:457: Bandeja:1 ↔ Remache POP Abierto con Rotura de Vástago D4:9
- Insert:458: Bandeja:1 ↔ Remache POP Abierto con Rotura de Vástago D4:11
- Insert:459: Remache POP Abierto con Rotura de Vástago D4:5 ↔ Bandeja:1
- Flush:41: Tornillo Gusano Allen M3x16mm:3 ↔ Tuerca de mesa:2
- Mate:344: Tornillo Gusano Allen M3x16mm:3 ↔ Tuerca de mesa:2
- Mate:345: Nema 17:2 ↔ NEMA 17 90°:1
- Mate:346: Nema 17:2 ↔ NEMA 17 90°:1
- Mate:347: Nema 17:2 ↔ NEMA 17 90°:1
- Mate:348: Columna Derecha:1 ↔ Estante para Soporte de Motor PaP:1
- Flush:42: Columna Derecha:1 ↔ Estante para Soporte de Motor PaP:1
- Mate:349: NEMA 17 90°:1 ↔ Estante para Soporte de Motor PaP:1
- Insert:465: Arandela Plana Tipo A DIN 125 - M4:3 ↔ Tornillo Allen cabeza cilindrica M4x20mm:7
- Mate:360: Chaponete:3 ↔ Arandela Plana Tipo A DIN 125 - M4:3
- Flush:49 (2.5 mm): Chaponete:3
- Mate:361: Tornillo Allen cabeza cilindrica M4x20mm:7
- Insert:466: Chaponete:3 ↔ Tornillo Allen cabeza fresada M3x20mm:4
- Flush:50 (-9 mm): Chaponete:3
- Mate:362: Tornillo Allen cabeza cilindrica M4x20mm:7
- Mate:363: Mesa:1 ↔ Tornillo Allen cabeza cilindrica M4x20mm:7
- Mate:364: Mesa:1 ↔ Chaponete:3
- Insert:467: Tornillo Allen cabeza cilindrica M4x20mm:9 ↔ Arandela Plana Tipo A DIN 125 - M4:5
- Mate:365: Chaponete:5 ↔ Arandela Plana Tipo A DIN 125 - M4:5
- Flush:51 (2.5 mm): Chaponete:5
- Flush:52 (-9 mm): Chaponete:5
- Insert:468: Chaponete:5 ↔ Tornillo Allen cabeza fresada M3x20mm:6
- Mate:366: Tornillo Allen cabeza cilindrica M4x20mm:9
- Mate:367: Tornillo Allen cabeza cilindrica M4x20mm:9
- Mate:368: Mesa:1 ↔ Tornillo Allen cabeza cilindrica M4x20mm:9
- Mate:369: Mesa:1 ↔ Chaponete:5
- Mate:370: Mesa:1 ↔ Tornillo Allen cabeza fresada M3x20mm:6
- Mate:371: Mesa:1 ↔ Tornillo Allen cabeza fresada M3x20mm:4
- Mate:372: Guía de Bandeja Izq.:1 ↔ Bandeja:1
- Mate:373: Remache POP Abierto con Rotura de Vástago D4:8 ↔ Guía de Bandeja Izq.:1
- Mate:374: Guía de Bandeja Der.:1 ↔ Esquina de bandeja:3
- Coincidencia:375 [Mate]: Frente Carcasa:1 ↔ Lateral Derecho Carcasa:1
- Coincidencia:376 [Mate]: Frente Carcasa:1 ↔ Lateral Derecho Carcasa:1
- Nivelación:53 [Flush]: Frente Carcasa:1 ↔ Lateral Derecho Carcasa:1
- Coincidencia:377 [Mate]: Frente Carcasa:1 ↔ Lateral Izquierdo Carcasa:1
- Coincidencia:378 [Mate]: Frente Carcasa:1 ↔ Lateral Izquierdo Carcasa:1
- Nivelación:54 [Flush]: Frente Carcasa:1 ↔ Lateral Izquierdo Carcasa:1
- Coincidencia:379 [Mate]: Lateral Derecho Carcasa:1 ↔ Techo Carcasa:1
- Nivelación:55 [Flush]: Lateral Derecho Carcasa:1 ↔ Techo Carcasa:1
- Nivelación:56 [Flush]: Lateral Derecho Carcasa:1 ↔ Techo Carcasa:1
- Coincidencia:380 [Mate]: Lateral Derecho Carcasa:1 ↔ Culata Carcaza:1
- Coincidencia:381 [Mate]: Lateral Derecho Carcasa:1 ↔ Culata Carcaza:1
- Coincidencia:382 [Mate]: Techo Carcasa:1 ↔ Culata Carcaza:1
- Insertar:469: Culata:1 ↔ Chapon:1
- Insertar:470: Culata:1 ↔ Chapon:1
- Coincidencia:383 [Mate]: Lateral:2 ↔ Separador Lateral:2
- Coincidencia:384 [Mate]: Columna Derecha:1 ↔ Separador Lateral:2
- Nivelación:57 [Flush]: Lateral:2 ↔ Separador Lateral:2
- Coincidencia:385 [Mate]: Lateral:1 ↔ Separador Lateral:1
- Nivelación:58 [Flush]: Lateral:1 ↔ Separador Lateral:1
- Coincidencia:386 [Mate]: Columna Izquierda:1 ↔ Separador Lateral:1
- Insertar:471: Lateral Derecho Carcasa:1 ↔ Cielo raso:1
- Insertar:472: Frente Carcasa:1 ↔ Cielo raso:1
- Coincidencia:387 [Mate]: Lateral Izquierdo Carcasa:1 ↔ Puerta Lateral Izquierda:1
- Coincidencia:388 [Mate]: Lateral Izquierdo Carcasa:1 ↔ Puerta Lateral Izquierda:1
- Coincidencia:389 [Mate]: Lateral Izquierdo Carcasa:1 ↔ Puerta Lateral Izquierda:1
- Insertar:473: Lateral Derecho Carcasa:1 ↔ Ala 1 Bisagra tipo Libro Grande:1
- Insertar:474: Lateral Derecho Carcasa:1 ↔ Ala 1 Bisagra tipo Libro Grande:1
- Insertar:475: Lateral Derecho Carcasa:1 ↔ Ala 1 Bisagra tipo Libro Grande:2
- Insertar:476: Lateral Derecho Carcasa:1 ↔ Ala 1 Bisagra tipo Libro Grande:2
- Insertar:477: Ala 1 Bisagra tipo Libro Grande:1 ↔ Ala 2 Bisagra tipo Libro Grande:1
- Insertar:478: Ala 1 Bisagra tipo Libro Grande:2 ↔ Ala 2 Bisagra tipo Libro Grande:2
- Coincidencia:392 [Mate]: Lateral Izquierdo Carcasa:1 ↔ Ala 1 Bisagra tipo T:1
- Insertar:481: Lateral Izquierdo Carcasa:1 ↔ Ala 1 Bisagra tipo T:1
- Coincidencia:393 [Mate]: Lateral Izquierdo Carcasa:1 ↔ Ala 1 Bisagra tipo T:1
- Coincidencia:394 [Mate]: Lateral Izquierdo Carcasa:1 ↔ Ala 1 Bisagra tipo T:2
- Insertar:482: Lateral Izquierdo Carcasa:1 ↔ Ala 1 Bisagra tipo T:2
- Coincidencia:395 [Mate]: Lateral Izquierdo Carcasa:1 ↔ Ala 1 Bisagra tipo T:2
- Insertar:483: Ala 1 Bisagra tipo T:1 ↔ Ala 2 Bisagra tipo T:1
- Insertar:484: Ala 1 Bisagra tipo T:2 ↔ Ala 2 Bisagra tipo T:2
- Insertar:487: Lateral:1 ↔ Distanciador para Laterales:3
- Insertar:488: Lateral:1 ↔ Distanciador para Laterales:2
- Insertar:489: Lateral:1 ↔ Distanciador para Laterales:1
- Insertar:490: Lateral:2 ↔ Distanciador para Laterales:6
- Insertar:491: Lateral:2 ↔ Distanciador para Laterales:5
- Insertar:492: Lateral:2 ↔ Distanciador para Laterales:4
- Coincidencia:396 [Mate]: Techo Carcasa:1 ↔ Ala 1 Bisagra tipo Libro Chica:2
- Insertar:493: Techo Carcasa:1 ↔ Ala 1 Bisagra tipo Libro Chica:2
- Coincidencia:397 [Mate]: Techo Carcasa:1 ↔ Ala 1 Bisagra tipo Libro Chica:2
- Coincidencia:398 [Mate]: Techo Carcasa:1 ↔ Ala 1 Bisagra tipo Libro Chica:1
- Insertar:494: Techo Carcasa:1 ↔ Ala 1 Bisagra tipo Libro Chica:1
- Coincidencia:399 [Mate]: Techo Carcasa:1 ↔ Ala 1 Bisagra tipo Libro Chica:1
- Insertar:495: Ala 1 Bisagra tipo Libro Chica:1 ↔ Ala 2 Bisagra tipo Libro Chica:1
- Coincidencia:400 [Mate]: Frente:1 ↔ Frente Carcasa:1
- Coincidencia:401 [Mate]: Lateral Izquierdo Carcasa:1 ↔ Distanciador para Laterales:2
- Coincidencia:402 [Mate]: Lateral Izquierdo Carcasa:1 ↔ Distanciador para Laterales:2
- Insertar:496: Ala 1 Bisagra tipo Libro Chica:2 ↔ Ala 2 Bisagra tipo Libro Chica:2
- Insertar:497: Soporte L:4 ↔ Tuerca remache m4:1
- Insertar:498: Soporte L:4 ↔ Tuerca remache m4:2
- Insertar:499: Soporte L:4 ↔ Tuerca remache m4:3
- Insertar:500: Soporte L:4 ↔ Tuerca remache m4:4
- Insertar:501: Soporte L:5 ↔ Tuerca remache m4:5
- Insertar:502: Soporte L:5 ↔ Tuerca remache m4:6
- Insertar:503: Soporte L:5 ↔ Tuerca remache m4:7
- Insertar:504: Soporte L:5 ↔ Tuerca remache m4:8
- Insertar:505: Soporte L:3 ↔ Tuerca remache m4:9
- Insertar:506: Soporte L:3 ↔ Tuerca remache m4:10
- Insertar:507: Soporte L:3 ↔ Tuerca remache m4:11
- Insertar:508: Soporte L:3 ↔ Tuerca remache m4:12
- Insertar:509: Soporte L:6 ↔ Tuerca remache m4:13
- Insertar:510: Soporte L:6 ↔ Tuerca remache m4:14
- Insertar:511: Soporte L:6 ↔ Tuerca remache m4:15
- Insertar:512: Soporte L:6 ↔ Tuerca remache m4:16
- Insertar:513: Soporte L:2 ↔ Tuerca remache m4:17
- Insertar:514: Soporte L:2 ↔ Tuerca remache m4:18
- Insertar:515: Soporte L:2 ↔ Tuerca remache m4:19
- Insertar:516: Soporte L:2 ↔ Tuerca remache m4:20
- Insertar:517: Soporte L:7 ↔ Tuerca remache m4:21
- Insertar:518: Soporte L:7 ↔ Tuerca remache m4:22
- Insertar:519: Soporte L:7 ↔ Tuerca remache m4:23
- Insertar:520: Soporte L:7 ↔ Tuerca remache m4:24
- Insertar:521: Soporte L:1 ↔ Tuerca remache m4:25
- Insertar:522: Soporte L:1 ↔ Tuerca remache m4:26
- Insertar:523: Soporte L:1 ↔ Tuerca remache m4:27
- Insertar:524: Soporte L:1 ↔ Tuerca remache m4:28
- Insertar:525: Soporte L:8 ↔ Tuerca remache m4:29
- Insertar:526: Soporte L:8 ↔ Tuerca remache m4:30
- Insertar:527: Soporte L:8 ↔ Tuerca remache m4:31
- Insertar:528: Soporte L:8 ↔ Tuerca remache m4:32
- Insertar:529: Lateral Derecho Carcasa:1 ↔ Tuerca remache m4:7
- Insertar:530: Lateral Derecho Carcasa:1 ↔ Tuerca remache m4:5
- Insertar:531: Lateral Derecho Carcasa:1 ↔ Tuerca remache m4:15
- Insertar:532: Lateral Derecho Carcasa:1 ↔ Tuerca remache m4:13
- Insertar:533: Lateral Izquierdo Carcasa:1 ↔ Tuerca remache m4:23
- Insertar:534: Lateral Izquierdo Carcasa:1 ↔ Tuerca remache m4:21
- Insertar:535: Lateral Izquierdo Carcasa:1 ↔ Tuerca remache m4:31
- Insertar:536: Lateral Izquierdo Carcasa:1 ↔ Tuerca remache m4:29
- Insertar:537: Techo Carcasa:1 ↔ Tuerca remache m4:28
- Insertar:538: Techo Carcasa:1 ↔ Tuerca remache m4:26
- Insertar:539: Lateral Izquierdo Carcasa:1 ↔ Tuerca remache m4:4
- Insertar:540: Lateral Izquierdo Carcasa:1 ↔ Tuerca remache m4:2
- Insertar:541: Lateral Derecho Carcasa:1 ↔ Tuerca remache m4:12
- Insertar:542: Lateral Derecho Carcasa:1 ↔ Tuerca remache m4:10
- Insertar:543: Frente Carcasa:1 ↔ Tuerca remache m4:17
- Insertar:544: Frente Carcasa:1 ↔ Tuerca remache m4:19
- Insertar:545: Lateral Izquierdo Carcasa:1 ↔ Chapa Base:1
- Insertar:546: Lateral Derecho Carcasa:1 ↔ Chapa Base:1
- Nivelación:59 [Flush]: Lateral Derecho Carcasa:1 ↔ Chapa Base:1
- Insertar:547: Tornillo Allen cabeza botón M6x20mm:41 ↔ Arandela plana tipo A DIN 125 M6:31
- Insertar:548: Tornillo Allen cabeza botón M6x20mm:42 ↔ Arandela plana tipo A DIN 125 M6:32
- Insertar:549: Tornillo Allen cabeza botón M6x20mm:43 ↔ Arandela plana tipo A DIN 125 M6:33
- Insertar:559: Tornillo Allen cabeza botón M6x20mm:53 ↔ Arandela plana tipo A DIN 125 M6:19
- Insertar:560: Tornillo Allen cabeza botón M6x20mm:54 ↔ Arandela plana tipo A DIN 125 M6:20
- Insertar:561: Tornillo Allen cabeza botón M6x20mm:55 ↔ Arandela plana tipo A DIN 125 M6:21
- Insertar:568: Lateral Derecho Carcasa:1 ↔ Arandela plana tipo A DIN 125 M6:31
- Insertar:569: Lateral Derecho Carcasa:1 ↔ Arandela plana tipo A DIN 125 M6:32
- Insertar:570: Lateral Derecho Carcasa:1 ↔ Arandela plana tipo A DIN 125 M6:33
- Insertar:571: Lateral Derecho Carcasa:1 ↔ Arandela plana tipo A DIN 125 M6:28
- Insertar:572: Lateral Derecho Carcasa:1 ↔ Arandela plana tipo A DIN 125 M6:29
- Insertar:573: Lateral Derecho Carcasa:1 ↔ Arandela plana tipo A DIN 125 M6:30
- Insertar:580: Lateral Izquierdo Carcasa:1 ↔ Arandela plana tipo A DIN 125 M6:19
- Insertar:581: Lateral Izquierdo Carcasa:1 ↔ Arandela plana tipo A DIN 125 M6:20
- Insertar:582: Lateral Izquierdo Carcasa:1 ↔ Arandela plana tipo A DIN 125 M6:21
- Insertar:583: Lateral Izquierdo Carcasa:1 ↔ Arandela plana tipo A DIN 125 M6:16
- Insertar:584: Lateral Izquierdo Carcasa:1 ↔ Arandela plana tipo A DIN 125 M6:17
- Insertar:585: Lateral Izquierdo Carcasa:1 ↔ Arandela plana tipo A DIN 125 M6:18
- Insertar:597: Tornillo Allen cabeza botón M4x20mm:7 ↔ Arandela Plana Tipo A DIN 125 - M4:18
- Insertar:598: Tornillo Allen cabeza botón M4x20mm:8 ↔ Arandela Plana Tipo A DIN 125 - M4:19
- Insertar:599: Tornillo Allen cabeza botón M4x20mm:9 ↔ Arandela Plana Tipo A DIN 125 - M4:20
- Insertar:600: Tornillo Allen cabeza botón M4x20mm:10 ↔ Arandela Plana Tipo A DIN 125 - M4:21
- Insertar:601: Tornillo Allen cabeza botón M4x20mm:11 ↔ Arandela Plana Tipo A DIN 125 - M4:23
- Insertar:602: Tornillo Allen cabeza botón M4x20mm:12 ↔ Arandela Plana Tipo A DIN 125 - M4:22
- Insertar:603: Tornillo Allen cabeza botón M4x20mm:13 ↔ Arandela Plana Tipo A DIN 125 - M4:24
- Insertar:604: Tornillo Allen cabeza botón M4x20mm:14 ↔ Arandela Plana Tipo A DIN 125 - M4:25
- Insertar:605: Tornillo Allen cabeza botón M4x20mm:15 ↔ Arandela Plana Tipo A DIN 125 - M4:33
- Insertar:606: Tornillo Allen cabeza botón M4x20mm:16 ↔ Arandela Plana Tipo A DIN 125 - M4:32
- Insertar:607: Tornillo Allen cabeza botón M4x20mm:17 ↔ Arandela Plana Tipo A DIN 125 - M4:31
- Insertar:608: Tornillo Allen cabeza botón M4x20mm:18 ↔ Arandela Plana Tipo A DIN 125 - M4:30
- Insertar:609: Tornillo Allen cabeza botón M4x20mm:19 ↔ Arandela Plana Tipo A DIN 125 - M4:29
- Insertar:610: Tornillo Allen cabeza botón M4x20mm:20 ↔ Arandela Plana Tipo A DIN 125 - M4:28
- Insertar:611: Tornillo Allen cabeza botón M4x20mm:21 ↔ Arandela Plana Tipo A DIN 125 - M4:27
- Insertar:612: Tornillo Allen cabeza botón M4x20mm:22 ↔ Arandela Plana Tipo A DIN 125 - M4:26
- Insertar:613: Tornillo Allen cabeza botón M4x20mm:23 ↔ Arandela Plana Tipo A DIN 125 - M4:34
- Insertar:614: Tornillo Allen cabeza botón M4x20mm:24 ↔ Arandela Plana Tipo A DIN 125 - M4:35
- Insertar:617: Tornillo Allen cabeza botón M4x20mm:27 ↔ Arandela Plana Tipo A DIN 125 - M4:38
- Insertar:618: Tornillo Allen cabeza botón M4x20mm:28 ↔ Arandela Plana Tipo A DIN 125 - M4:39
- Insertar:619: Tornillo Allen cabeza botón M4x20mm:29 ↔ Arandela Plana Tipo A DIN 125 - M4:40
- Insertar:620: Tornillo Allen cabeza botón M4x20mm:30 ↔ Arandela Plana Tipo A DIN 125 - M4:41
- Insertar:621: Lateral Derecho Carcasa:1 ↔ Arandela Plana Tipo A DIN 125 - M4:18
- Insertar:622: Culata Carcaza:1 ↔ Arandela Plana Tipo A DIN 125 - M4:19
- Insertar:623: Culata Carcaza:1 ↔ Arandela Plana Tipo A DIN 125 - M4:20
- Insertar:624: Lateral Derecho Carcasa:1 ↔ Arandela Plana Tipo A DIN 125 - M4:21
- Insertar:625: Lateral Derecho Carcasa:1 ↔ Arandela Plana Tipo A DIN 125 - M4:23
- Insertar:626: Culata Carcaza:1 ↔ Arandela Plana Tipo A DIN 125 - M4:22
- Insertar:627: Culata Carcaza:1 ↔ Arandela Plana Tipo A DIN 125 - M4:24
- Insertar:628: Lateral Derecho Carcasa:1 ↔ Arandela Plana Tipo A DIN 125 - M4:25
- Insertar:629: Lateral Derecho Carcasa:1 ↔ Arandela Plana Tipo A DIN 125 - M4:33
- Insertar:630: Techo Carcasa:1 ↔ Arandela Plana Tipo A DIN 125 - M4:32
- Insertar:631: Techo Carcasa:1 ↔ Arandela Plana Tipo A DIN 125 - M4:31
- Insertar:632: Lateral Derecho Carcasa:1 ↔ Arandela Plana Tipo A DIN 125 - M4:30
- Insertar:633: Techo Carcasa:1 ↔ Arandela Plana Tipo A DIN 125 - M4:29
- Insertar:634: Culata Carcaza:1 ↔ Arandela Plana Tipo A DIN 125 - M4:28
- Insertar:635: Techo Carcasa:1 ↔ Arandela Plana Tipo A DIN 125 - M4:27
- Insertar:636: Culata Carcaza:1 ↔ Arandela Plana Tipo A DIN 125 - M4:26
- Insertar:637: Lateral Derecho Carcasa:1 ↔ Arandela Plana Tipo A DIN 125 - M4:41
- Insertar:638: Lateral Derecho Carcasa:1 ↔ Arandela Plana Tipo A DIN 125 - M4:40
- Insertar:639: Frente Carcasa:1 ↔ Arandela Plana Tipo A DIN 125 - M4:39
- Insertar:640: Frente Carcasa:1 ↔ Arandela Plana Tipo A DIN 125 - M4:38
- Insertar:641: Tornillo Allen cabeza botón M4x20mm:31 ↔ Arandela Plana Tipo A DIN 125 - M4:6
- Insertar:642: Tornillo Allen cabeza botón M4x20mm:32 ↔ Arandela Plana Tipo A DIN 125 - M4:7
- Insertar:643: Tornillo Allen cabeza botón M4x20mm:33 ↔ Arandela Plana Tipo A DIN 125 - M4:8
- Insertar:644: Tornillo Allen cabeza botón M4x20mm:34 ↔ Arandela Plana Tipo A DIN 125 - M4:9
- Insertar:645: Tornillo Allen cabeza botón M4x20mm:35 ↔ Arandela Plana Tipo A DIN 125 - M4:10
- Insertar:646: Tornillo Allen cabeza botón M4x20mm:36 ↔ Arandela Plana Tipo A DIN 125 - M4:11
- Insertar:647: Tornillo Allen cabeza botón M4x20mm:37 ↔ Arandela Plana Tipo A DIN 125 - M4:12